# Autodesk Inventor assembly: Assembled
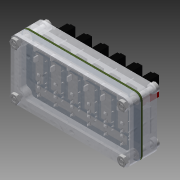
[picture p0: Inventor's stored thumbnail of the model, 180x180]
Saved by Autodesk Inventor 2014 SP1 (Build 180222100, 222)
## iProperties
Created: 2016-03-18
Part Number: Assembled
Document SubType Name: Assembly
Designer: Tyler
Author: Tyler
## Documents named in this file (8)
- C:\Users\Tyler\Documents\powerpolebreakout\Cad\Assembled.iam
- C:\Users\Tyler\Documents\powerpolebreakout\Cad\PopulatedPCB.iam
- C:\Users\Tyler\Documents\powerpolebreakout\Cad\AcrylicUpperCore.ipt
- C:\Users\Tyler\Documents\powerpolebreakout\Cad\AcrylicUpperTop.ipt
- C:\Users\Tyler\Documents\powerpolebreakout\Cad\AcrylicLowerCore.ipt
- C:\Users\Tyler\Documents\powerpolebreakout\Cad\AcrylicLowerBottom.ipt
- C:\Users\Tyler\Documents\Inventor\Content Center Files\R2014\en-US\AS 1112 (4)\AS 1112 - M4(2).ipt
- C:\Users\Tyler\Documents\Inventor\Content Center Files\R2014\en-US\AS 1420\AS 1420 - 1973 - M4 x 25.ipt
## Components (13 placed, 7 different names)
1. PopulatedPCB:1 [sub-assembly] — Flush:1, Flush:2, Mate:1, Flush:5, Flush:6, Mate:3
2. AcrylicUpperCore:1 — Flush:1, Flush:2, Mate:1, Flush:3, Flush:4, Mate:2, Mate:6
3. AcrylicUpperTop:1 — Flush:3, Flush:4, Mate:2, Mate:5, Insert:1, Insert:2, Insert:3
4. AcrylicLowerCore:1 — Flush:5, Flush:6, Mate:3, Flush:7, Flush:8, Mate:4
5. AcrylicLowerBottom:1 — Flush:7, Flush:8, Mate:4, Mate:7, Mate:10, Mate:11, Mate:14
6. AS 1420 - Metric M4 x 25:3 — Mate:5, Mate:6, Mate:13
7. AS 1420 - Metric M4 x 25:4 — Insert:1, Mate:12
8. AS 1420 - Metric M4 x 25:2 — Insert:2, Mate:9
9. AS 1420 - Metric M4 x 25:1 — Insert:3, Mate:8
10. AS 1112 (4) - Metric M4:1 — Mate:7, Mate:8
11. AS 1112 (4) - Metric M4:2 — Mate:9, Mate:10
12. AS 1112 (4) - Metric M4:3 — Mate:13, Mate:14
13. AS 1112 (4) - Metric M4:4 — Mate:11, Mate:12
## Relationships (25: Mate 14, Flush 8, Insert 3)
- Flush:1: PopulatedPCB:1 ↔ AcrylicUpperCore:1
- Flush:2: PopulatedPCB:1 ↔ AcrylicUpperCore:1
- Mate:1: PopulatedPCB:1 ↔ AcrylicUpperCore:1
- Flush:3: AcrylicUpperCore:1 ↔ AcrylicUpperTop:1
- Flush:4: AcrylicUpperCore:1 ↔ AcrylicUpperTop:1
- Mate:2: AcrylicUpperCore:1 ↔ AcrylicUpperTop:1
- Flush:5: PopulatedPCB:1 ↔ AcrylicLowerCore:1
- Flush:6: PopulatedPCB:1 ↔ AcrylicLowerCore:1
- Mate:3: PopulatedPCB:1 ↔ AcrylicLowerCore:1
- Flush:7: AcrylicLowerCore:1 ↔ AcrylicLowerBottom:1
- Flush:8: AcrylicLowerCore:1 ↔ AcrylicLowerBottom:1
- Mate:4: AcrylicLowerCore:1 ↔ AcrylicLowerBottom:1
- Mate:5: AcrylicUpperTop:1 ↔ AS 1420 - Metric M4 x 25:3
- Mate:6: AcrylicUpperCore:1 ↔ AS 1420 - Metric M4 x 25:3
- Insert:1: AcrylicUpperTop:1 ↔ AS 1420 - Metric M4 x 25:4
- Insert:2: AcrylicUpperTop:1 ↔ AS 1420 - Metric M4 x 25:2
- Insert:3: AcrylicUpperTop:1 ↔ AS 1420 - Metric M4 x 25:1
- Mate:7: AcrylicLowerBottom:1 ↔ AS 1112 (4) - Metric M4:1
- Mate:8: AS 1420 - Metric M4 x 25:1 ↔ AS 1112 (4) - Metric M4:1
- Mate:9: AS 1420 - Metric M4 x 25:2 ↔ AS 1112 (4) - Metric M4:2
- Mate:10: AcrylicLowerBottom:1 ↔ AS 1112 (4) - Metric M4:2
- Mate:11: AcrylicLowerBottom:1 ↔ AS 1112 (4) - Metric M4:4
- Mate:12: AS 1420 - Metric M4 x 25:4 ↔ AS 1112 (4) - Metric M4:4
- Mate:13: AS 1420 - Metric M4 x 25:3 ↔ AS 1112 (4) - Metric M4:3
- Mate:14: AcrylicLowerBottom:1 ↔ AS 1112 (4) - Metric M4:3
